# Autodesk Inventor assembly: piece_asm
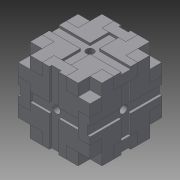
[picture p0: Inventor's stored thumbnail of the model, 180x180]
Saved by Autodesk Inventor 2015 (Build 190159000, 159)
## iProperties
Created: 2017-11-05
Part Number: piece_asm
Document SubType Name: Assembly
Designer: tasuku
Author: tasuku
## Documents named in this file (2)
- C:\Users\tasuku\Documents\cnc_text\test_part\piece_asm.iam
- C:\Users\tasuku\Documents\cnc_text\test_part\piece_1.ipt
## Components (6 placed, 1 different names)
1. piece_1:1 — フラッシュ:1, フラッシュ:2, フラッシュ:3, フラッシュ:4, フラッシュ:6, フラッシュ:9, フラッシュ:10
2. piece_1:2 — フラッシュ:1, フラッシュ:2, フラッシュ:3, フラッシュ:5, フラッシュ:11, フラッシュ:12
3. piece_1:3 — フラッシュ:4, フラッシュ:5, フラッシュ:6, フラッシュ:7, フラッシュ:8
4. piece_1:4 — フラッシュ:7, フラッシュ:8, フラッシュ:9, フラッシュ:13, フラッシュ:15
5. piece_1:5 — フラッシュ:10, フラッシュ:11, フラッシュ:12, フラッシュ:14
6. piece_1:6 — フラッシュ:13, フラッシュ:14, フラッシュ:15
## Relationships (15: Flush 15)
- フラッシュ:1 [Flush]: piece_1:1 ↔ piece_1:2
- フラッシュ:2 [Flush]: piece_1:1 ↔ piece_1:2
- フラッシュ:3 [Flush]: piece_1:1 ↔ piece_1:2
- フラッシュ:4 [Flush]: piece_1:1 ↔ piece_1:3
- フラッシュ:5 [Flush]: piece_1:2 ↔ piece_1:3
- フラッシュ:6 [Flush]: piece_1:1 ↔ piece_1:3
- フラッシュ:7 [Flush]: piece_1:3 ↔ piece_1:4
- フラッシュ:8 [Flush]: piece_1:3 ↔ piece_1:4
- フラッシュ:9 [Flush]: piece_1:1 ↔ piece_1:4
- フラッシュ:10 [Flush]: piece_1:1 ↔ piece_1:5
- フラッシュ:11 [Flush]: piece_1:2 ↔ piece_1:5
- フラッシュ:12 [Flush]: piece_1:2 ↔ piece_1:5
- フラッシュ:13 [Flush]: piece_1:4 ↔ piece_1:6
- フラッシュ:14 [Flush]: piece_1:5 ↔ piece_1:6
- フラッシュ:15 [Flush]: piece_1:4 ↔ piece_1:6
